# Autodesk Inventor assembly: UpperArm_MIR_without_bumper
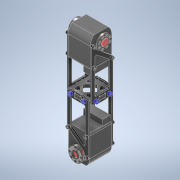
[picture p0: Inventor's stored thumbnail of the model, 180x180]
Saved by Autodesk Inventor 2022 (Build 260153000, 153)
## iProperties
Created: 2021-09-11
Part Number: UpperArm_MIR_without_bumper
Document SubType Name: Assembly
Designer: Masato Kubotera
Mass: 132.402 g
Surface Area: 432.665 cm^2
Volume: 110.152 cm^3
Density: 1.20199 g/cm^3
Author: Masato
## Documents named in this file (7)
- C:\Users\MasatoKubotera\Documents\Inventor\SUSTAINA-OP\UpperBody\Arm\UpperArm_MIR_without_bumper.iam
- C:\Users\MasatoKubotera\Documents\Inventor\SUSTAINA-OP\UpperBody\Arm\UpperArm_diagonal.iam
- C:\Users\MasatoKubotera\Documents\Inventor\SUSTAINA-OP\UpperBody\Arm\UpperArm_side_frame.ipt
- C:\Users\MasatoKubotera\Documents\Inventor\SUSTAINA-OP\ReadyMade\KONDO\B3M-SC-1040-A_with_ClampHorn_AND_FreeHorn.iam
- C:\Users\MasatoKubotera\Documents\Inventor\SUSTAINA-OP\ReadyMade\Screw\UC-0306.ipt
- C:\Users\MasatoKubotera\Documents\Inventor\SUSTAINA-OP\ReadyMade\Screw\FC-2615EB.ipt
- C:\Users\MasatoKubotera\Documents\Inventor\SUSTAINA-OP\ReadyMade\Screw\FC-2620EB.ipt
## Components (27 placed, 6 different names)
1. UpperArm_diagonal:1 [sub-assembly] — Insert:93, Insert:92, Insert:91, Insert:90, Insert:89, Insert:88, Insert:87, Insert:86
2. UpperArm_side_frame:1 — Insert:85, Insert:84, Insert:34, Insert:33, Insert:32, Insert:80, Insert:75, Insert:74, Insert:89, Insert:88
3. UpperArm_side_frame:2 — Insert:40, 挿入:39, 挿入:38, Insert:12, Insert:11, Insert:83, Insert:82, Insert:81, Insert:93, Insert:92
4. UpperArm_side_frame:3 — Insert:37, Insert:36, Insert:35, Insert:13, Insert:14, Insert:79, Insert:78, Insert:77, Insert:87, Insert:86
5. UpperArm_side_frame:4 — Insert:31, Insert:30, Insert:29, Insert:16, Insert:15, Insert:76, Insert:73, Insert:72, Insert:91, Insert:90
6. B3M-SC-1040-A_with_ClampHorn_AND_FreeHorn:1 [sub-assembly] — Insert:79, Insert:78, Insert:77, Insert:76, Insert:73, Insert:72
7. B3M-SC-1040-A_with_ClampHorn_AND_FreeHorn:2 [sub-assembly] — Insert:83, Insert:82, Insert:81, Insert:80, Insert:75, Insert:74
8. UC-0306:1 — Insert:85
9. UC-0306:2 — Insert:11
10. UC-0306:3 — Insert:12
11. UC-0306:4 — Insert:13
12. UC-0306:5 — Insert:14
13. UC-0306:6 — Insert:15
14. UC-0306:7 — Insert:16
15. FC-2615EB:1 — Insert:31
16. FC-2615EB:2 — Insert:32
17. FC-2615EB:3 — Insert:33
18. FC-2615EB:4 — Insert:34
19. UC-0306:8 — Insert:84
20. FC-2615EB:5 — Insert:29
21. FC-2615EB:6 — Insert:30
22. FC-2620EB:1 — Insert:37
23. FC-2620EB:2 — 挿入:39
24. FC-2620EB:3 — 挿入:38
25. FC-2620EB:4 — Insert:40
26. FC-2620EB:5 — Insert:35
27. FC-2620EB:6 — Insert:36
## Relationships (40: Insert 40)
- Insert:37: UpperArm_side_frame:3 ↔ FC-2620EB:1
- Insert:36: UpperArm_side_frame:3 ↔ FC-2620EB:6
- Insert:35: UpperArm_side_frame:3 ↔ FC-2620EB:5
- Insert:13: UpperArm_side_frame:3 ↔ UC-0306:4
- Insert:14: UpperArm_side_frame:3 ↔ UC-0306:5
- Insert:31: UpperArm_side_frame:4 ↔ FC-2615EB:1
- Insert:30: UpperArm_side_frame:4 ↔ FC-2615EB:6
- Insert:29: UpperArm_side_frame:4 ↔ FC-2615EB:5
- Insert:16: UpperArm_side_frame:4 ↔ UC-0306:7
- Insert:15: UpperArm_side_frame:4 ↔ UC-0306:6
- Insert:85: UpperArm_side_frame:1 ↔ UC-0306:1
- Insert:84: UpperArm_side_frame:1 ↔ UC-0306:8
- Insert:34: UpperArm_side_frame:1 ↔ FC-2615EB:4
- Insert:33: UpperArm_side_frame:1 ↔ FC-2615EB:3
- Insert:32: UpperArm_side_frame:1 ↔ FC-2615EB:2
- Insert:40: UpperArm_side_frame:2 ↔ FC-2620EB:4
- 挿入:39 [Insert]: UpperArm_side_frame:2 ↔ FC-2620EB:2
- 挿入:38 [Insert]: UpperArm_side_frame:2 ↔ FC-2620EB:3
- Insert:12: UpperArm_side_frame:2 ↔ UC-0306:3
- Insert:11: UpperArm_side_frame:2 ↔ UC-0306:2
- Insert:79: UpperArm_side_frame:3 ↔ B3M-SC-1040-A_with_ClampHorn_AND_FreeHorn:1
- Insert:78: UpperArm_side_frame:3 ↔ B3M-SC-1040-A_with_ClampHorn_AND_FreeHorn:1
- Insert:77: UpperArm_side_frame:3 ↔ B3M-SC-1040-A_with_ClampHorn_AND_FreeHorn:1
- Insert:76: UpperArm_side_frame:4 ↔ B3M-SC-1040-A_with_ClampHorn_AND_FreeHorn:1
- Insert:73: UpperArm_side_frame:4 ↔ B3M-SC-1040-A_with_ClampHorn_AND_FreeHorn:1
- Insert:72: UpperArm_side_frame:4 ↔ B3M-SC-1040-A_with_ClampHorn_AND_FreeHorn:1
- Insert:83: UpperArm_side_frame:2 ↔ B3M-SC-1040-A_with_ClampHorn_AND_FreeHorn:2
- Insert:82: UpperArm_side_frame:2 ↔ B3M-SC-1040-A_with_ClampHorn_AND_FreeHorn:2
- Insert:81: UpperArm_side_frame:2 ↔ B3M-SC-1040-A_with_ClampHorn_AND_FreeHorn:2
- Insert:80: UpperArm_side_frame:1 ↔ B3M-SC-1040-A_with_ClampHorn_AND_FreeHorn:2
- Insert:75: UpperArm_side_frame:1 ↔ B3M-SC-1040-A_with_ClampHorn_AND_FreeHorn:2
- Insert:74: UpperArm_side_frame:1 ↔ B3M-SC-1040-A_with_ClampHorn_AND_FreeHorn:2
- Insert:93: UpperArm_diagonal:1 ↔ UpperArm_side_frame:2
- Insert:92: UpperArm_diagonal:1 ↔ UpperArm_side_frame:2
- Insert:91: UpperArm_diagonal:1 ↔ UpperArm_side_frame:4
- Insert:90: UpperArm_diagonal:1 ↔ UpperArm_side_frame:4
- Insert:89: UpperArm_diagonal:1 ↔ UpperArm_side_frame:1
- Insert:88: UpperArm_diagonal:1 ↔ UpperArm_side_frame:1
- Insert:87: UpperArm_diagonal:1 ↔ UpperArm_side_frame:3
- Insert:86: UpperArm_diagonal:1 ↔ UpperArm_side_frame:3
